# Autodesk Inventor assembly: SSCMN4
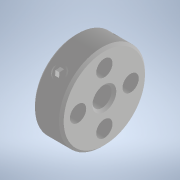
[picture p0: Inventor's stored thumbnail of the model, 180x180]
Saved by Autodesk Inventor 2021 (Build 250183000, 183)
## iProperties
Category: PARTsolutions
Company: MISUMI
Created: 2025-03-10
Part Number: SSCMN4
Catalog Web Link: www.cadenas.de
Description: SCMN, PSCMN, SSCMN-Shaft Collars - with Holes - 4 Holes
Vendor: MISUMI
Document SubType Name: Assembly
Designer: psAdmin
Manufacturer: MISUMI
Mass: 1.18184 g
Surface Area: 12.1881 cm^2
Volume: 1.18184 cm^3
Density: 1 g/cm^3
Title: SSCMN4
Author: Cadenas PARTsolutions
Comments: Shaft Collars - with Holes - 4 Holes
PSOL_IDENT_0: {$CADENAS_DATA/23d-libs/misumi/metric/03_set_collars/scmn_asmtab.prj},184 {VTYP=3D},{STYP=ASSTAB},{N
PSOL_IDENT_1: B=SSCMN4},{LINA=SSCMN4},{NN=SCMN, PSCMN, SSCMN},{DATE=02.06.2021 02:59:54},{GEOMDATE=25.12.2015 06:0
PSOL_IDENT_2: 8:42},{VERSION=},{LINEID=20},{WBVAR=MAT,ST},{WBNUMERIC=}  {NB=SSCMN4},{LINA=SSCMN4},{KT=DUMMY},{PN=S
PSOL_IDENT_3: SCMN4},{TYPE=SSCMN},{MAT=304},{ST=-},{AC=Set Screws 2 Pcs. (304 Stainless Steel) },{D=4},{B=6},{D1=1
PSOL_IDENT_4: 8},{S=3.4},{P=11},{M=M3x3},{THMD=3},{THDMIN=2.459},{C=0.5},{ST0='-','-'},{L=3},{PPATH=scmn/scmn_temp
PSOL_IDENT_5: l.prj}
NB: SSCMN4
NN: SCMN, PSCMN, SSCMN
NT: Shaft Collars - with Holes - 4 Holes
NBSYN: $PN.
LINA: SSCMN4
CATALOG: Misumi
PN: SSCMN4
MAT: SUS304 Equivalent
ST: -
AC: Set Screws 2 Pcs. (304 Stainless Steel)
D: 4
B: 6
D1: 18
S: 3.4
P: 11
M: M3x3
SUPPLIER: MISUMI
ARTICLENO: SSCMN4
BOMINFO: SSCMN4
CREATOR: CADENAS GmbH
## Documents named in this file (3)
- e:\temp\worker_COMMON_119\temp\tmp_8724_272_p2WT5\format_0\SSCMN4.iam
- e:\temp\worker_COMMON_119\temp\tmp_8724_272_p2WT5\format_0\SSCMN4b.ipt
- e:\temp\worker_COMMON_119\temp\tmp_8724_272_p2WT5\format_0\Hexagon socket set screw with flat point DIN 913 - M3x3.ipt
## Components (3 placed, 2 different names)
1. SSCMN4b:1 — body_set_v_Z@1 <-> IP1_Z@2, body_set_h_Z@1 <-> IP1_Z@3
2. Hexagon socket set screw with flat point DIN 913 - M3x3:1 — body_set_v_Z@1 <-> IP1_Z@2
3. Hexagon socket set screw with flat point DIN 913 - M3x3:2 — body_set_h_Z@1 <-> IP1_Z@3
## Relationships (2: Mate 2)
- body_set_v_Z@1 <-> IP1_Z@2 [Mate]: SSCMN4b:1 ↔ Hexagon socket set screw with flat point DIN 913 - M3x3:1
- body_set_h_Z@1 <-> IP1_Z@3 [Mate]: SSCMN4b:1 ↔ Hexagon socket set screw with flat point DIN 913 - M3x3:2
